# Autodesk Inventor assembly: pallet_step
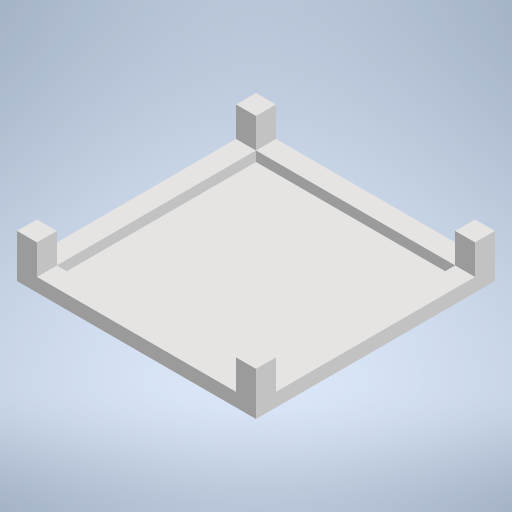
[picture p0: Inventor's stored thumbnail of the model, 512x512]
Saved by Autodesk Inventor 2024 (Build 280153000, 153)
## iProperties
Created: 2024-01-12
Part Number: pallet_step
Document SubType Name: Assembly
Designer: nicky
Author: nicky
## Documents named in this file (4)
- D:\OneDrive - 성균관대학교\Projects\2024 ICRA QRC 대회\모델\pallet_step.iam
- D:\OneDrive - 성균관대학교\Projects\2024 ICRA QRC 대회\모델\board_18x1200x1200.ipt
- D:\OneDrive - 성균관대학교\Projects\2024 ICRA QRC 대회\모델\board_50x100x1200.ipt
- D:\OneDrive - 성균관대학교\Projects\2024 ICRA QRC 대회\모델\board_100x100x150.ipt
## Components (9 placed, 3 different names)
1. board_18x1200x1200:1 — 플러쉬:1, 메이트:2, 메이트:3, 플러쉬:2, 플러쉬:3, 메이트:4, 플러쉬:7
2. board_50x100x1200:1 — 플러쉬:1, 플러쉬:4, 플러쉬:5, 플러쉬:6, 메이트:6, 플러쉬:13
3. board_50x100x1200:3 — 메이트:2, 플러쉬:4, 플러쉬:5, 플러쉬:8, 메이트:5, 플러쉬:9, 플러쉬:10
4. board_50x100x1200:4 — 메이트:3, 플러쉬:2, 플러쉬:3, 플러쉬:11
5. board_50x100x1200:5 — 메이트:4, 플러쉬:6, 플러쉬:7, 메이트:7, 플러쉬:12, 플러쉬:14
6. board_100x100x150:1 — 플러쉬:8
7. board_100x100x150:2 — 메이트:5, 플러쉬:9, 플러쉬:10
8. board_100x100x150:3 — 메이트:6, 플러쉬:13, 플러쉬:14
9. board_100x100x150:4 — 메이트:7, 플러쉬:11, 플러쉬:12
## Relationships (20: Flush 14, Mate 6)
- 플러쉬:1 [Flush]: board_18x1200x1200:1 ↔ board_50x100x1200:1
- 메이트:2 [Mate]: board_18x1200x1200:1 ↔ board_50x100x1200:3
- 메이트:3 [Mate]: board_18x1200x1200:1 ↔ board_50x100x1200:4
- 플러쉬:2 [Flush]: board_18x1200x1200:1 ↔ board_50x100x1200:4
- 플러쉬:3 [Flush]: board_18x1200x1200:1 ↔ board_50x100x1200:4
- 플러쉬:4 [Flush]: board_50x100x1200:1 ↔ board_50x100x1200:3
- 플러쉬:5 [Flush]: board_50x100x1200:1 ↔ board_50x100x1200:3
- 메이트:4 [Mate]: board_18x1200x1200:1 ↔ board_50x100x1200:5
- 플러쉬:6 [Flush]: board_50x100x1200:1 ↔ board_50x100x1200:5
- 플러쉬:7 [Flush]: board_18x1200x1200:1 ↔ board_50x100x1200:5
- 플러쉬:8 [Flush]: board_50x100x1200:3 ↔ board_100x100x150:1
- 메이트:5 [Mate]: board_50x100x1200:3 ↔ board_100x100x150:2
- 메이트:6 [Mate]: board_50x100x1200:1 ↔ board_100x100x150:3
- 메이트:7 [Mate]: board_50x100x1200:5 ↔ board_100x100x150:4
- 플러쉬:9 [Flush]: board_50x100x1200:3 ↔ board_100x100x150:2
- 플러쉬:10 [Flush]: board_50x100x1200:3 ↔ board_100x100x150:2
- 플러쉬:11 [Flush]: board_50x100x1200:4 ↔ board_100x100x150:4
- 플러쉬:12 [Flush]: board_50x100x1200:5 ↔ board_100x100x150:4
- 플러쉬:13 [Flush]: board_50x100x1200:1 ↔ board_100x100x150:3
- 플러쉬:14 [Flush]: board_50x100x1200:5 ↔ board_100x100x150:3
